# Autodesk Inventor assembly: MMBOT
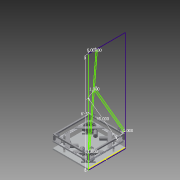
[picture p0: Inventor's stored thumbnail of the model, 180x180]
Saved by Autodesk Inventor 2013 SP2 (Build 170200200, 200)
## iProperties
Created: 2015-01-07
Part Number: MMBOT
Document SubType Name: Assembly
Designer: darkb_000
Author: darkb_000
## Documents named in this file (25)
- C:\Users\Public\Documents\Autodesk\Vault Basic 2013\Samples\Inventor 2013\Padlock\Designs\MMBOT.iam
- C:\Users\darkb_000\Desktop\BotLayoutGLass.ipt
- C:\Users\Public\Documents\Autodesk\Vault Basic 2013\Samples\Inventor 2013\Padlock\Designs\LibraryMG\Chassis\Chassis_AndyMark_am-0453\Cchannel27inch.ipt
- C:\Users\Public\Documents\Autodesk\Vault Basic 2013\Samples\Inventor 2013\Padlock\Designs\LibraryMG\Chassis\Chassis_AndyMark_am-0453\Chassis_Channel_26_AndyMark_am-0202.ipt
- C:\Users\Public\Documents\Autodesk\Vault Basic 2013\Samples\Inventor 2013\Padlock\Designs\LibraryMG\Chassis\Chassis_AndyMark_am-0453\Chassis_CornerConnect_AndyMark_am-0212.ipt
- C:\Users\Public\Documents\Autodesk\Vault Basic 2013\Samples\Inventor 2013\Padlock\Designs\HolonomicCornerBracket.ipt
- C:\Users\Public\Documents\Autodesk\Vault Basic 2013\Samples\Inventor 2013\Padlock\Designs\HolonomicCornerBracket02.ipt
- C:\Users\Public\Documents\Autodesk\Vault Basic 2013\Samples\Inventor 2013\Padlock\Designs\LibraryMG\Gears\Imported Components\Toughbox-nano-500-key-long-asm\Toughbox-nano-500-key-long-asm.iam
- C:\Users\Public\Documents\Autodesk\Vault Basic 2013\Samples\Inventor 2013\Padlock\Designs\LibraryMG\Wheels\Imported Components\8-Molded-Trick-Wheel\8-Molded-Trick-Wheel.iam
- C:\Users\Public\Documents\Autodesk\Vault Basic 2013\Samples\Inventor 2013\Padlock\Designs\HolonomicCornerBracket_MIR.ipt
- C:\Users\Public\Documents\Autodesk\Vault Basic 2013\Samples\Inventor 2013\Padlock\Designs\HolonomicCornerBracket02_MIR.ipt
- C:\Users\Public\Documents\Autodesk\Vault Basic 2013\Samples\Inventor 2013\Padlock\Designs\LibraryMG\Gears\Imported Components\Toughbox-nano-500-key-long-asm\Toughbox-nano-500-key-long-asm_MIR.iam
- C:\Users\Public\Documents\Autodesk\Vault Basic 2013\Samples\Inventor 2013\Padlock\Designs\LibraryMG\Wheels\Imported Components\8-Molded-Trick-Wheel\8-Molded-Trick-Wheel_MIR.iam
- C:\Users\Public\Documents\Autodesk\Vault Basic 2013\Samples\Inventor 2013\Padlock\Designs\HolonomicCornerBracket_MIR1.ipt
- C:\Users\Public\Documents\Autodesk\Vault Basic 2013\Samples\Inventor 2013\Padlock\Designs\HolonomicCornerBracket02_MIR1.ipt
- C:\Users\Public\Documents\Autodesk\Vault Basic 2013\Samples\Inventor 2013\Padlock\Designs\LibraryMG\Gears\Imported Components\Toughbox-nano-500-key-long-asm\Toughbox-nano-500-key-long-asm_MIR1.iam
- C:\Users\Public\Documents\Autodesk\Vault Basic 2013\Samples\Inventor 2013\Padlock\Designs\LibraryMG\Wheels\Imported Components\8-Molded-Trick-Wheel\8-Molded-Trick-Wheel_MIR1.iam
- C:\Users\Public\Documents\Autodesk\Vault Basic 2013\Samples\Inventor 2013\Padlock\Designs\HolonomicCornerBracket_MIR_MIR.ipt
- C:\Users\Public\Documents\Autodesk\Vault Basic 2013\Samples\Inventor 2013\Padlock\Designs\HolonomicCornerBracket02_MIR_MIR.ipt
- C:\Users\Public\Documents\Autodesk\Vault Basic 2013\Samples\Inventor 2013\Padlock\Designs\LibraryMG\Gears\Imported Components\Toughbox-nano-500-key-long-asm\Toughbox-nano-500-key-long-asm_MIR_MIR.iam
- C:\Users\Public\Documents\Autodesk\Vault Basic 2013\Samples\Inventor 2013\Padlock\Designs\LibraryMG\Wheels\Imported Components\8-Molded-Trick-Wheel\8-Molded-Trick-Wheel_MIR_MIR.iam
- C:\Users\Public\Documents\Autodesk\Vault Basic 2013\Samples\Inventor 2013\Padlock\Designs\3inchUp.ipt
- C:\Users\Public\Documents\Autodesk\Vault Basic 2013\Samples\Inventor 2013\Padlock\Designs\SideLong.ipt
- C:\Users\Public\Documents\Autodesk\Vault Basic 2013\Samples\Inventor 2013\Padlock\Designs\backlong.ipt
- C:\Users\Public\Documents\Autodesk\Vault Basic 2013\Samples\Inventor 2013\Padlock\Designs\LibraryMG\Chassis\Chassis_AndyMark_am-0453\channelBracket02.ipt
## Components (37 placed, 24 different names)
1. BotLayoutGLass:1 — Flush:1, Flush:2, Flush:4, Mate:19
2. Cchannel27inch:1 — Flush:1, Flush:2, Flush:5, Mate:1, Mate:2, Mate:5, Mate:7, Mate:8, Flush:7, Mate:19, Flush:10, Flush:11
3. Cchannel27inch:2 — Flush:4, Flush:5, Mate:13, Mate:14, Mate:15, Mate:16
4. Chassis_Channel_26_AndyMark_am-0202:1 — Mate:9, Mate:10, Flush:7, Mate:17, Mate:18
5. Chassis_Channel_26_AndyMark_am-0202:2 — Mate:3, Mate:4, Mate:6, Mate:11, Mate:12
6. Chassis_CornerConnect_AndyMark_am-0212:1 — Mate:11, Mate:12, Mate:13, Mate:14, Flush:8, Flush:9
7. Chassis_CornerConnect_AndyMark_am-0212:2 — Mate:15, Mate:16, Mate:17, Mate:18, Flush:9
8. Chassis_CornerConnect_AndyMark_am-0212:3 — Mate:7, Mate:8, Mate:9, Mate:10, Flush:6
9. Chassis_CornerConnect_AndyMark_am-0212:4 — Mate:1, Mate:2, Mate:3, Mate:4, Mate:5, Mate:6, Flush:6, Flush:8
10. HolonomicCornerBracket:1 — Flush:10, Mate:23, Mate:36, Flush:17, Flush:18
11. HolonomicCornerBracket02:1 — Flush:11, Mate:20, Mate:21, Flush:12
12. Toughbox-nano-500-key-long-asm:1 [sub-assembly] — Mate:20, Mate:21, Flush:12, Mate:22
13. 8-Molded-Trick-Wheel:1 [sub-assembly] — Mate:22, Mate:23
14. HolonomicCornerBracket_MIR:1 — Mate:26, Flush:16
15. HolonomicCornerBracket02_MIR:1 — Flush:13, Mate:24, Mate:25
16. Toughbox-nano-500-key-long-asm_MIR:1 [sub-assembly] — Flush:13, Mate:24, Mate:25, Mate:27
17. 8-Molded-Trick-Wheel_MIR:1 [sub-assembly] — Mate:26, Mate:27
18. HolonomicCornerBracket_MIR1:1 — Mate:30, Mate:37, Flush:19, Flush:20
19. HolonomicCornerBracket02_MIR1:1 — Flush:14, Mate:28, Mate:29
20. Toughbox-nano-500-key-long-asm_MIR1:1 [sub-assembly] — Flush:14, Mate:28, Mate:29, Mate:31
21. 8-Molded-Trick-Wheel_MIR1:1 [sub-assembly] — Mate:30, Mate:31
22. HolonomicCornerBracket_MIR_MIR:1 — Mate:35, Mate:38, Flush:21, Flush:22
23. HolonomicCornerBracket02_MIR_MIR:1 — Mate:32, Mate:33, Flush:15
24. Toughbox-nano-500-key-long-asm_MIR_MIR:1 [sub-assembly] — Mate:32, Mate:33, Flush:15, Mate:34
25. 8-Molded-Trick-Wheel_MIR_MIR:1 [sub-assembly] — Mate:34, Mate:35
26. 3inchUp:1 — Flush:16, Flush:27
27. 3inchUp:2 — Mate:36, Flush:17, Flush:18, Flush:24, Flush:25, Mate:39
28. 3inchUp:3 — Mate:37, Flush:19, Flush:20
29. 3inchUp:4 — Mate:38, Flush:21, Flush:22, Flush:23
30. SideLong:1 — Flush:23, Flush:26, Mate:40, Flush:28
31. SideLong:2 — Flush:24, Flush:25, Mate:39, Flush:31
32. backlong:1 — Flush:26, Mate:45, Mate:46, Mate:47, Mate:48
33. backlong:2 — Mate:40, Flush:27, Flush:28, Mate:41, Mate:42, Mate:43, Mate:44
34. channelBracket02:1 — Mate:43, Mate:44, Flush:29, Mate:49
35. channelBracket02:2 — Mate:41, Mate:42, Flush:30, Mate:49, Flush:31
36. channelBracket02:3 — Mate:45, Mate:46, Flush:30
37. channelBracket02:4 — Mate:47, Mate:48, Flush:29
## Relationships (79: Mate 49, Flush 30)
- Flush:1: BotLayoutGLass:1 ↔ Cchannel27inch:1
- Flush:2: BotLayoutGLass:1 ↔ Cchannel27inch:1
- Flush:4: BotLayoutGLass:1 ↔ Cchannel27inch:2
- Flush:5: Cchannel27inch:1 ↔ Cchannel27inch:2
- Mate:1: Cchannel27inch:1 ↔ Chassis_CornerConnect_AndyMark_am-0212:4
- Mate:2: Cchannel27inch:1 ↔ Chassis_CornerConnect_AndyMark_am-0212:4
- Mate:3: Chassis_Channel_26_AndyMark_am-0202:2 ↔ Chassis_CornerConnect_AndyMark_am-0212:4
- Mate:4: Chassis_Channel_26_AndyMark_am-0202:2 ↔ Chassis_CornerConnect_AndyMark_am-0212:4
- Mate:5: Cchannel27inch:1 ↔ Chassis_CornerConnect_AndyMark_am-0212:4
- Mate:6: Chassis_Channel_26_AndyMark_am-0202:2 ↔ Chassis_CornerConnect_AndyMark_am-0212:4
- Mate:7: Cchannel27inch:1 ↔ Chassis_CornerConnect_AndyMark_am-0212:3
- Mate:8: Cchannel27inch:1 ↔ Chassis_CornerConnect_AndyMark_am-0212:3
- Mate:9: Chassis_Channel_26_AndyMark_am-0202:1 ↔ Chassis_CornerConnect_AndyMark_am-0212:3
- Mate:10: Chassis_Channel_26_AndyMark_am-0202:1 ↔ Chassis_CornerConnect_AndyMark_am-0212:3
- Flush:6: Chassis_CornerConnect_AndyMark_am-0212:3 ↔ Chassis_CornerConnect_AndyMark_am-0212:4
- Flush:7: Cchannel27inch:1 ↔ Chassis_Channel_26_AndyMark_am-0202:1
- Mate:11: Chassis_Channel_26_AndyMark_am-0202:2 ↔ Chassis_CornerConnect_AndyMark_am-0212:1
- Mate:12: Chassis_Channel_26_AndyMark_am-0202:2 ↔ Chassis_CornerConnect_AndyMark_am-0212:1
- Mate:13: Cchannel27inch:2 ↔ Chassis_CornerConnect_AndyMark_am-0212:1
- Mate:14: Cchannel27inch:2 ↔ Chassis_CornerConnect_AndyMark_am-0212:1
- Flush:8: Chassis_CornerConnect_AndyMark_am-0212:1 ↔ Chassis_CornerConnect_AndyMark_am-0212:4
- Mate:15: Cchannel27inch:2 ↔ Chassis_CornerConnect_AndyMark_am-0212:2
- Mate:16: Cchannel27inch:2 ↔ Chassis_CornerConnect_AndyMark_am-0212:2
- Mate:17: Chassis_Channel_26_AndyMark_am-0202:1 ↔ Chassis_CornerConnect_AndyMark_am-0212:2
- Mate:18: Chassis_Channel_26_AndyMark_am-0202:1 ↔ Chassis_CornerConnect_AndyMark_am-0212:2
- Flush:9: Chassis_CornerConnect_AndyMark_am-0212:1 ↔ Chassis_CornerConnect_AndyMark_am-0212:2
- Mate:19 (101.6 mm): BotLayoutGLass:1 ↔ Cchannel27inch:1
- Flush:10: Cchannel27inch:1 ↔ HolonomicCornerBracket:1
- Flush:11: Cchannel27inch:1 ↔ HolonomicCornerBracket02:1
- Mate:20: HolonomicCornerBracket02:1 ↔ Toughbox-nano-500-key-long-asm:1
- Mate:21: HolonomicCornerBracket02:1 ↔ Toughbox-nano-500-key-long-asm:1
- Flush:12: HolonomicCornerBracket02:1 ↔ Toughbox-nano-500-key-long-asm:1
- Mate:22: Toughbox-nano-500-key-long-asm:1 ↔ 8-Molded-Trick-Wheel:1
- Mate:23 (25.4 mm): HolonomicCornerBracket:1 ↔ 8-Molded-Trick-Wheel:1
- Flush:13: HolonomicCornerBracket02_MIR:1 ↔ Toughbox-nano-500-key-long-asm_MIR:1
- Mate:24: HolonomicCornerBracket02_MIR:1 ↔ Toughbox-nano-500-key-long-asm_MIR:1
- Mate:25: HolonomicCornerBracket02_MIR:1 ↔ Toughbox-nano-500-key-long-asm_MIR:1
- Mate:26 (25.4 mm): HolonomicCornerBracket_MIR:1 ↔ 8-Molded-Trick-Wheel_MIR:1
- Mate:27: Toughbox-nano-500-key-long-asm_MIR:1 ↔ 8-Molded-Trick-Wheel_MIR:1
- Flush:14: HolonomicCornerBracket02_MIR1:1 ↔ Toughbox-nano-500-key-long-asm_MIR1:1
- Mate:28: HolonomicCornerBracket02_MIR1:1 ↔ Toughbox-nano-500-key-long-asm_MIR1:1
- Mate:29: HolonomicCornerBracket02_MIR1:1 ↔ Toughbox-nano-500-key-long-asm_MIR1:1
- Mate:30 (25.4 mm): HolonomicCornerBracket_MIR1:1 ↔ 8-Molded-Trick-Wheel_MIR1:1
- Mate:31: Toughbox-nano-500-key-long-asm_MIR1:1 ↔ 8-Molded-Trick-Wheel_MIR1:1
- Mate:32: HolonomicCornerBracket02_MIR_MIR:1 ↔ Toughbox-nano-500-key-long-asm_MIR_MIR:1
- Mate:33: HolonomicCornerBracket02_MIR_MIR:1 ↔ Toughbox-nano-500-key-long-asm_MIR_MIR:1
- Flush:15: HolonomicCornerBracket02_MIR_MIR:1 ↔ Toughbox-nano-500-key-long-asm_MIR_MIR:1
- Mate:34: Toughbox-nano-500-key-long-asm_MIR_MIR:1 ↔ 8-Molded-Trick-Wheel_MIR_MIR:1
- Mate:35 (25.4 mm): HolonomicCornerBracket_MIR_MIR:1 ↔ 8-Molded-Trick-Wheel_MIR_MIR:1
- Flush:16: HolonomicCornerBracket_MIR:1 ↔ 3inchUp:1
- Mate:36: HolonomicCornerBracket:1 ↔ 3inchUp:2
- Flush:17: HolonomicCornerBracket:1 ↔ 3inchUp:2
- Flush:18: HolonomicCornerBracket:1 ↔ 3inchUp:2
- Mate:37: HolonomicCornerBracket_MIR1:1 ↔ 3inchUp:3
- Flush:19: HolonomicCornerBracket_MIR1:1 ↔ 3inchUp:3
- Flush:20: HolonomicCornerBracket_MIR1:1 ↔ 3inchUp:3
- Mate:38: HolonomicCornerBracket_MIR_MIR:1 ↔ 3inchUp:4
- Flush:21: HolonomicCornerBracket_MIR_MIR:1 ↔ 3inchUp:4
- Flush:22: HolonomicCornerBracket_MIR_MIR:1 ↔ 3inchUp:4
- Flush:23: 3inchUp:4 ↔ SideLong:1
- Flush:24: 3inchUp:2 ↔ SideLong:2
- Flush:25: 3inchUp:2 ↔ SideLong:2
- Mate:39: 3inchUp:2 ↔ SideLong:2
- Flush:26: SideLong:1 ↔ backlong:1
- Mate:40: SideLong:1 ↔ backlong:2
- Flush:27: 3inchUp:1 ↔ backlong:2
- Flush:28: SideLong:1 ↔ backlong:2
- Mate:41: backlong:2 ↔ channelBracket02:2
- Mate:42: backlong:2 ↔ channelBracket02:2
- Mate:43: backlong:2 ↔ channelBracket02:1
- Mate:44: backlong:2 ↔ channelBracket02:1
- Mate:45: backlong:1 ↔ channelBracket02:3
- Mate:46: backlong:1 ↔ channelBracket02:3
- Mate:47: backlong:1 ↔ channelBracket02:4
- Mate:48: backlong:1 ↔ channelBracket02:4
- Flush:29: channelBracket02:1 ↔ channelBracket02:4
- Flush:30: channelBracket02:2 ↔ channelBracket02:3
- Mate:49 (457.2 mm): channelBracket02:1 ↔ channelBracket02:2
- Flush:31 (-82.55 mm): SideLong:2 ↔ channelBracket02:2
